# Autodesk Inventor assembly: tower
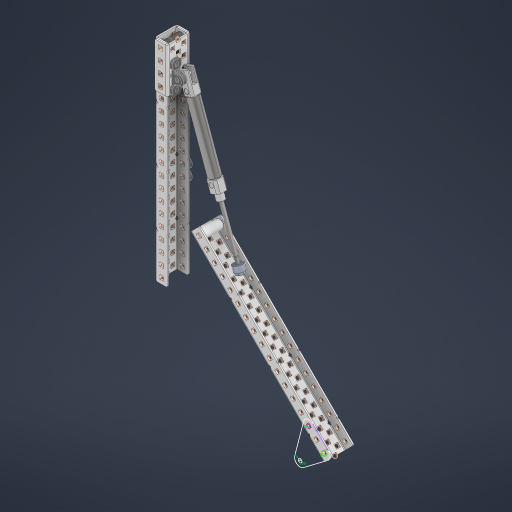
[picture p0: Inventor's stored thumbnail of the model, 512x512]
Saved by Autodesk Inventor 2024 (Build 280153000, 153)
## iProperties
Created: 2024-01-16
Part Number: tower
Document SubType Name: Assembly
Designer: avere
Author: avere
## Documents named in this file (16)
- C:\Users\avere\Documents\rbp_cad\zoomba_v0.3\tower\side.iam
- C:\Users\avere\Documents\rbp_cad\VEX-CAD-Inventor-1.41\Structure\C Channel\Aluminum 1x2x1\Alu C 1x2x1x19.ipt
- C:\Users\avere\Documents\rbp_cad\VEX-CAD-Inventor-1.41\Structure\C Channel\Aluminum 1x2x1\Alu C 1x2x1x4.ipt
- C:\Users\avere\Documents\rbp_cad\VEX-CAD-Inventor-1.41\Motion\Spacers\Spacer Nylon .500 OD\NSpacer Black .500 OD x .125.ipt
- C:\Users\avere\Documents\rbp_cad\VEX-CAD-Inventor-1.41\Motion\Spacers\Spacer Nylon .500 OD.ipt
- C:\Users\avere\Documents\rbp_cad\VEX-CAD-Inventor-1.41\Motion\Shaft LS\LS Pillow Bearing Block.ipt
- C:\Users\avere\Documents\rbp_cad\VEX-CAD-Inventor-1.41\Motion\Spacers\Spacer Nylon .375 OD\NSpacer .375 OD x .250.ipt
- C:\Users\avere\Documents\rbp_cad\VEX-CAD-Inventor-1.41\Motion\Spacers\Spacer Nylon .375 OD.ipt
- C:\Users\avere\Documents\rbp_cad\VEX-CAD-Inventor-1.41\Motion\Spacers\Spacer Nylon .375 OD\NSpacer .375 OD x .500.ipt
- C:\Users\avere\Documents\rbp_cad\VEX-CAD-Inventor-1.41\Motion\Spacers\Washer Steel\SWasher .375 OD x .062500.ipt
- C:\Users\avere\Documents\rbp_cad\VEX-CAD-Inventor-1.41\Motion\Spacers\Washer Steel.ipt
- C:\Users\avere\Documents\rbp_cad\VEX-CAD-Inventor-1.41\Motion\Pneumatics\Double Acting Piston.iam
- C:\Users\avere\Documents\rbp_cad\VEX-CAD-Inventor-1.41\Structure\C Channel\Aluminum 1x2x1\Alu C 1x2x1x17.ipt
- C:\Users\avere\Documents\rbp_cad\VEX-CAD-Inventor-1.41\Motion\Shaft LS\Shaft Collar ipts\Shaft Collar No Screw.ipt
- C:\Users\avere\Documents\rbp_cad\VEX-CAD-Inventor-1.41\Motion\Pneumatics\Piston Nut.ipt
- C:\Users\avere\Documents\rbp_cad\hardware\.375 OD Aluminum Spacer 0.875.ipt
## Components (13 placed, 12 different names)
1. Alu C 1x2x1x19:2 — Insert:3, Insert:4, Angle:1
2. Alu C 1x2x1x4:1 — Insert:5, Mate:2, Insert:8
3. NSpacer Black .500 OD x .125:3 — Insert:4
4. NSpacer Black .500 OD x .125:4 — Insert:3
5. LS Pillow Bearing Block:1 — Insert:5, Mate:2, Insert:9
6. NSpacer .375 OD x .250:1 — Insert:6, Insert:7
7. NSpacer .375 OD x .500:2 — Insert:7, Insert:8
8. SWasher .375 OD x .062500:1 — Insert:6
9. Double Acting Piston:1 [sub-assembly] — Insert:9, Insert:11
10. Alu C 1x2x1x17:1 — Mate:3, Angle:1, Insert:12
11. Shaft Collar No Screw:1 — Mate:3
12. Piston Nut:1 — Insert:11
13. .375 OD Aluminum Spacer 0.875:1 — Insert:12
## Relationships (15: Insert 11, Mate 3, Angle 1)
- [Insert]: Alu C 1x2x1x19:2 ↔ Alu C 1x2x1x4:1
- [Mate]: Alu C 1x2x1x19:2 ↔ Alu C 1x2x1x4:1
- Insert:3: Alu C 1x2x1x19:2 ↔ NSpacer Black .500 OD x .125:4
- Insert:4: Alu C 1x2x1x19:2 ↔ NSpacer Black .500 OD x .125:3
- Insert:5 (1.5875 mm): Alu C 1x2x1x4:1 ↔ LS Pillow Bearing Block:1
- Mate:2: Alu C 1x2x1x4:1 ↔ LS Pillow Bearing Block:1
- Insert:6: NSpacer .375 OD x .250:1 ↔ SWasher .375 OD x .062500:1
- Insert:7: NSpacer .375 OD x .250:1 ↔ NSpacer .375 OD x .500:2
- Insert:8: Alu C 1x2x1x4:1 ↔ NSpacer .375 OD x .500:2
- Insert:9: LS Pillow Bearing Block:1 ↔ Double Acting Piston:1
- [Insert]: Shaft Collar No Screw:1 ↔ Piston Nut:1
- Insert:11: Double Acting Piston:1 ↔ Piston Nut:1
- Mate:3: Alu C 1x2x1x17:1 ↔ Shaft Collar No Screw:1
- Angle:1 (0 deg): Alu C 1x2x1x19:2 ↔ Alu C 1x2x1x17:1
- Insert:12: Alu C 1x2x1x17:1 ↔ .375 OD Aluminum Spacer 0.875:1
